# Autodesk Inventor assembly: Neck_Cover_United
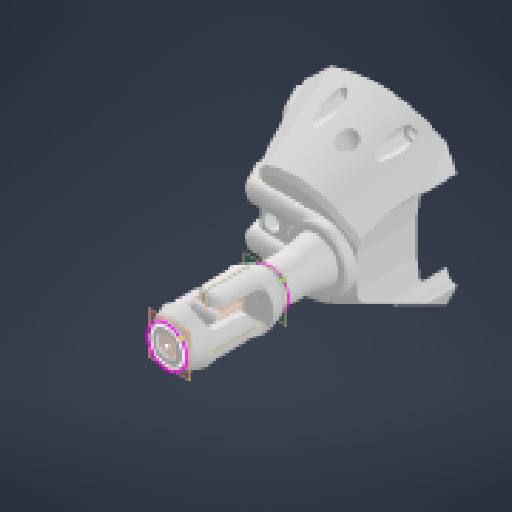
[picture p0: Inventor's stored thumbnail of the model, 512x512]
Saved by Autodesk Inventor 2024 (Build 280153000, 153)
## iProperties
Created: 2025-09-27
Part Number: Neck_Cover_United
Document SubType Name: Assembly
Designer: kevin
Author: kevin
## Documents named in this file (3)
- C:\Users\kevin\Desktop\SeniorDesign\Head_V3\Neck_Cover_United.iam
- C:\Users\kevin\Desktop\Neck_Cover.ipt
- C:\Users\kevin\Desktop\SeniorDesign\Universal_Joint.iam
## Components (2 placed, 2 different names)
1. Neck_Cover:1 — Mate:1, Mate:2
2. Universal_Joint:1 [sub-assembly] — Mate:1, Mate:2
## Relationships (2: Mate 2)
- Mate:1: Neck_Cover:1 ↔ Universal_Joint:1
- Mate:2: Neck_Cover:1 ↔ Universal_Joint:1
